# Autodesk Inventor assembly: laser circle assembly
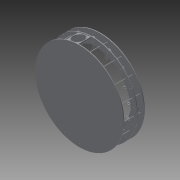
[picture p0: Inventor's stored thumbnail of the model, 180x180]
Saved by Autodesk Inventor 2013 (Build 170138000, 138)
## iProperties
Created: 2013-07-18
Part Number: laser circle assembly
Document SubType Name: Assembly
Designer: owner
Author: owner
## Documents named in this file (7)
- C:\Users\owner\Dropbox\EDW Harp\laser circle assembly.iam
- C:\Users\owner\Dropbox\EDW Harp\laser circle 3D.ipt
- C:\Users\owner\Dropbox\EDW Harp\laser supports.ipt
- C:\Users\owner\Dropbox\EDW Harp\speakermount.ipt
- C:\Users\owner\Dropbox\EDW Harp\laser circle3d back.ipt
- C:\Users\owner\Dropbox\EDW Harp\standoffs.ipt
- C:\Users\Public\Documents\Autodesk\Vault Basic 2013\Samples\Inventor 2013\Padlock\Designs\back layer of front.ipt
## Components (37 placed, 6 different names)
1. laser circle 3D:1 — Insert:1, Mate:1, Mate:2, Mate:3, Mate:4
2. speakermount:1 — Mate:3, Mate:4, Mate:5, Mate:6
3. speakermount:2 — Mate:1, Mate:2
4. laser circle3d back:1 — Mate:5, Mate:6, Insert:2
5. back layer of front:1 — Insert:3
6. laser supports:1 — Insert:1
7. laser supports:2
8. laser supports:3
9. laser supports:4
10. laser supports:5
11. laser supports:6
12. laser supports:7
13. laser supports:8
14. laser supports:9
15. laser supports:10
16. laser supports:11
17. laser supports:12
18. laser supports:13
19. laser supports:14
20. laser supports:15
21. laser supports:16
22. laser supports:17
23. standoffs:1 — Insert:2
24. standoffs:2
25. standoffs:3 — Insert:3
26. standoffs:4
27. standoffs:6
28. standoffs:7
29. standoffs:8
30. standoffs:9
31. standoffs:10
32. standoffs:11
33. standoffs:12
34. standoffs:14
35. standoffs:15
36. standoffs:16
37. standoffs:17
## Component patterns: (17 elements, first: laser supports:1), (17 elements, first: standoffs:1)
## Relationships (9: Mate 6, Insert 3)
- Insert:1: laser circle 3D:1 ↔ laser supports:1
- Mate:1: laser circle 3D:1 ↔ speakermount:2
- Mate:2: laser circle 3D:1 ↔ speakermount:2
- Mate:3: laser circle 3D:1 ↔ speakermount:1
- Mate:4: laser circle 3D:1 ↔ speakermount:1
- Mate:5: speakermount:1 ↔ laser circle3d back:1
- Mate:6: speakermount:1 ↔ laser circle3d back:1
- Insert:2: laser circle3d back:1 ↔ standoffs:1
- Insert:3: back layer of front:1 ↔ standoffs:3
